# Autodesk Inventor assembly: 足回り
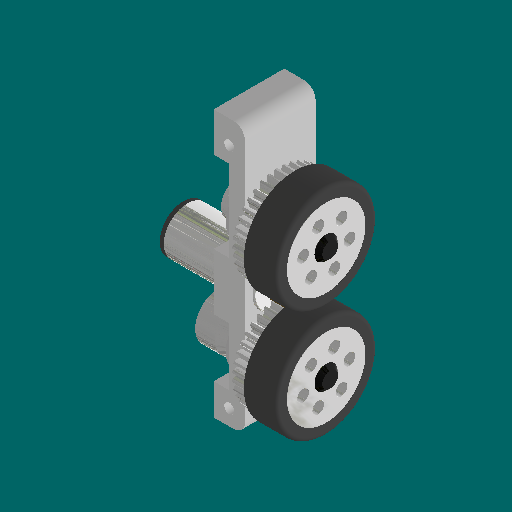
[picture p0: Inventor's stored thumbnail of the model, 512x512]
Saved by Autodesk Inventor 2023 (Build 270158000, 158)
## iProperties
Created: 2022-03-31
Part Number: 足回り
Document SubType Name: Assembly
Designer: neko2
Author: neko2
## Documents named in this file (12)
- C:\Users\hide\Desktop\SaponseEx\CAD\足回り.iam
- C:\Users\hide\Desktop\SaponseEx\CAD\FL673ZZ.ipt
- C:\Users\hide\Desktop\SaponseEx\CAD\HeikoPin.ipt
- C:\Users\hide\Desktop\SaponseEx\CAD\RT-PN v2.ipt
- C:\Users\hide\Desktop\SaponseEx\CAD\Tire.ipt
- C:\Users\hide\Desktop\SaponseEx\CAD\Stopper.ipt
- C:\Users\hide\Desktop\SaponseEx\CAD\Magnet.iam
- C:\Users\hide\Desktop\SaponseEx\CAD\Magnet_Simple.ipt
- C:\Users\hide\Desktop\SaponseEx\CAD\Magnet.ipt
- C:\Users\hide\Desktop\SaponseEx\CAD\Gear.iam
- C:\Users\hide\Desktop\SaponseEx\CAD\CoreLessMotor.ipt
- C:\Users\hide\Desktop\SaponseEx\CAD\MotorMount_New.ipt
## Components (17 placed, 10 different names)
1. CoreLessMotor:1 — 回転:1, リジッド:31
2. FL673ZZ:1 — メイト:29, リジッド:33
3. FL673ZZ:2 — リジッド:34, 円柱状:22, メイト:36
4. FL673ZZ:3 — リジッド:35, メイト:37
5. FL673ZZ:4 — メイト:32, リジッド:32, 円柱状:21
6. HeikoPin:1 — 円柱状:17, 円柱状:19, リジッド:28, 円柱状:22
7. HeikoPin:2 — 円柱状:18, 円柱状:20, 円柱状:21, メイト:38
8. RT-PN v2:1 — 回転:1
9. Tire:1 — リジッド:30
10. Tire:2 — リジッド:29
11. Stopper:1 — 円柱状:18, メイト:29
12. Magnet:1 [sub-assembly] — 円柱状:17
13. Magnet_Simple:1 — 円柱状:19, リジッド:27, メイト:37
14. Magnet:2 — リジッド:27
15. Gear:1 [sub-assembly] — 円柱状:20, メイト:32, リジッド:30, メイト:38
16. Gear:2 [sub-assembly] — リジッド:28, リジッド:29, メイト:36
17. MotorMount_New:1 — メイト:34, フラッシュ:36, メイト:35, リジッド:31, リジッド:32, リジッド:33, リジッド:34, リジッド:35
## Relationships (24: WeldJoint 9, Mate 7, CylindricalJoint 6, RevoluteJoint 1, Flush 1)
- 円柱状:17 [CylindricalJoint]: HeikoPin:1 ↔ Magnet:1
- 円柱状:18 [CylindricalJoint]: HeikoPin:2 ↔ Stopper:1
- メイト:29 [Mate]: FL673ZZ:1 ↔ Stopper:1
- 円柱状:19 [CylindricalJoint]: HeikoPin:1 ↔ Magnet_Simple:1
- リジッド:27 [WeldJoint]: Magnet_Simple:1 ↔ Magnet:2
- 円柱状:20 [CylindricalJoint]: HeikoPin:2 ↔ Gear:1
- メイト:32 [Mate]: FL673ZZ:4 ↔ Gear:1
- リジッド:28 [WeldJoint]: HeikoPin:1 ↔ Gear:2
- リジッド:29 [WeldJoint]: Tire:2 ↔ Gear:2
- リジッド:30 [WeldJoint]: Tire:1 ↔ Gear:1
- 回転:1 [RevoluteJoint] (0.2 mm): CoreLessMotor:1 ↔ RT-PN v2:1
- メイト:34 [Mate]: MotorMount_New:1
- フラッシュ:36 [Flush]: MotorMount_New:1
- メイト:35 [Mate]: MotorMount_New:1
- リジッド:31 [WeldJoint]: CoreLessMotor:1 ↔ MotorMount_New:1
- リジッド:32 [WeldJoint]: FL673ZZ:4 ↔ MotorMount_New:1
- リジッド:33 [WeldJoint]: FL673ZZ:1 ↔ MotorMount_New:1
- 円柱状:21 [CylindricalJoint]: FL673ZZ:4 ↔ HeikoPin:2
- リジッド:34 [WeldJoint]: FL673ZZ:2 ↔ MotorMount_New:1
- リジッド:35 [WeldJoint]: FL673ZZ:3 ↔ MotorMount_New:1
- 円柱状:22 [CylindricalJoint]: FL673ZZ:2 ↔ HeikoPin:1
- メイト:36 [Mate]: FL673ZZ:2 ↔ Gear:2
- メイト:37 [Mate]: FL673ZZ:3 ↔ Magnet_Simple:1
- メイト:38 [Mate]: HeikoPin:2 ↔ Gear:1
